# Autodesk Inventor assembly: LM2596 DC-DC Buck Converter Module
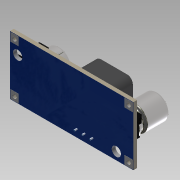
[picture p0: Inventor's stored thumbnail of the model, 180x180]
Saved by Autodesk Inventor 2019 (Build 230136000, 136)
## iProperties
Created: 2019-03-04
Part Number: LM2596 DC-DC Buck Converter Module
Document SubType Name: Assembly
Designer: ZEUSLAP
Author: ZEUSLAP
## Documents named in this file (11)
- C:\Users\Luis Pujol\Desktop\AURA MODELADO\ELECTRONICA\AURA ELECTRONICA\LM2596 DC-DC Buck Converter Module.iam
- LM2596 DC-DC Buck Converter Module.iam
- C:\Users\Luis Pujol\Dropbox\TRABAJO\DISEÑO MECANICO Y PRESUPUESTOS\CAJAS PROYECTOS\PROYECTO 1\LM2596\parts\trimpot.ipt
- C:\Users\Luis Pujol\Dropbox\TRABAJO\DISEÑO MECANICO Y PRESUPUESTOS\CAJAS PROYECTOS\PROYECTO 1\LM2596\parts\board.ipt
- C:\Users\Luis Pujol\Dropbox\TRABAJO\DISEÑO MECANICO Y PRESUPUESTOS\CAJAS PROYECTOS\PROYECTO 1\LM2596\parts\capacitor.ipt
- C:\Users\Luis Pujol\Dropbox\TRABAJO\DISEÑO MECANICO Y PRESUPUESTOS\CAJAS PROYECTOS\PROYECTO 1\LM2596\parts\CAPSMD220-35.ipt
- C:\Users\Luis Pujol\Dropbox\TRABAJO\DISEÑO MECANICO Y PRESUPUESTOS\CAJAS PROYECTOS\PROYECTO 1\LM2596\parts\Diode SMA.ipt
- C:\Users\Luis Pujol\Dropbox\TRABAJO\DISEÑO MECANICO Y PRESUPUESTOS\CAJAS PROYECTOS\PROYECTO 1\LM2596\parts\inductor.ipt
- C:\Users\Luis Pujol\Dropbox\TRABAJO\DISEÑO MECANICO Y PRESUPUESTOS\CAJAS PROYECTOS\PROYECTO 1\LM2596\parts\lm2596.ipt
- C:\Users\Luis Pujol\Dropbox\TRABAJO\DISEÑO MECANICO Y PRESUPUESTOS\CAJAS PROYECTOS\PROYECTO 1\LM2596\parts\resistor.ipt
- C:\Users\Luis Pujol\Dropbox\TRABAJO\DISEÑO MECANICO Y PRESUPUESTOS\CAJAS PROYECTOS\PROYECTO 1\LM2596\parts\solder_hole.ipt
## Components (13 placed, 9 different names)
1. board:1 — Mate:1, Mate:2, Mate:3, Mate:4, Mate:5, Mate:6, Mate:7, Mate:8, Mate:9, Mate:10, Angle:1, Mate:11, Angle:2, Mate:12, Angle:3, Mate:13, Angle:4, Angle:5, Angle:6, Mate:14, Mate:15, Mate:16, Mate:17, Mate:18, Mate:19, Mate:20, Mate:21, Mate:22, Mate:28, Mate:29
2. capacitor:1 — Mate:7, Angle:5, Mate:30, Mate:31
3. CAPSMD220-35:1 — Mate:3, Angle:3, Mate:13, Mate:28, Mate:31
4. Diode SMA:1 — Mate:5, Angle:4, Mate:22, Mate:23
5. inductor:1 — Mate:2, Mate:26, Mate:27, Mate:30
6. lm2596:1 — Mate:1, Angle:1, Mate:11, Mate:24, Mate:25, Mate:27
7. resistor:1 — Mate:8, Angle:6, Mate:29, Flush:1
8. trimpot:1 — Mate:6, Angle:2, Mate:12, Mate:25, Mate:26, Flush:1
9. CAPSMD220-35:2 — Mate:4, Mate:9, Mate:10, Mate:23, Mate:24
10. solder_hole:1 — Mate:18, Mate:19
11. solder_hole:2 — Mate:14, Mate:15
12. solder_hole:3 — Mate:16, Mate:17
13. solder_hole:4 — Mate:20, Mate:21
## Relationships (38: Mate 31, Angle 6, Flush 1)
- Mate:1: board:1 ↔ lm2596:1
- Mate:2: board:1 ↔ inductor:1
- Mate:3: board:1 ↔ CAPSMD220-35:1
- Mate:4: board:1 ↔ CAPSMD220-35:2
- Mate:5: board:1 ↔ Diode SMA:1
- Mate:6: board:1 ↔ trimpot:1
- Mate:7: board:1 ↔ capacitor:1
- Mate:8: board:1 ↔ resistor:1
- Mate:9: board:1 ↔ CAPSMD220-35:2
- Mate:10: board:1 ↔ CAPSMD220-35:2
- Angle:1 (0 deg): board:1 ↔ lm2596:1
- Mate:11: board:1 ↔ lm2596:1
- Angle:2 (-90 deg): board:1 ↔ trimpot:1
- Mate:12: board:1 ↔ trimpot:1
- Angle:3 (0 deg): board:1 ↔ CAPSMD220-35:1
- Mate:13: board:1 ↔ CAPSMD220-35:1
- Angle:4 (180 deg): board:1 ↔ Diode SMA:1
- Angle:5 (90 deg): board:1 ↔ capacitor:1
- Angle:6 (0 deg): board:1 ↔ resistor:1
- Mate:14: board:1 ↔ solder_hole:2
- Mate:15: board:1 ↔ solder_hole:2
- Mate:16: board:1 ↔ solder_hole:3
- Mate:17: board:1 ↔ solder_hole:3
- Mate:18: board:1 ↔ solder_hole:1
- Mate:19: board:1 ↔ solder_hole:1
- Mate:20: board:1 ↔ solder_hole:4
- Mate:21: board:1 ↔ solder_hole:4
- Mate:22 (3.5 mm): board:1 ↔ Diode SMA:1
- Mate:23 (2 mm): Diode SMA:1 ↔ CAPSMD220-35:2
- Mate:24 (0.5 mm): lm2596:1 ↔ CAPSMD220-35:2
- Mate:25 (0.5 mm): lm2596:1 ↔ trimpot:1
- Mate:26 (0.5 mm): inductor:1 ↔ trimpot:1
- Mate:27 (0.3 mm): inductor:1 ↔ lm2596:1
- Mate:28 (6 mm): board:1 ↔ CAPSMD220-35:1
- Mate:29 (1.5 mm): board:1 ↔ resistor:1
- Flush:1 (-2 mm): resistor:1 ↔ trimpot:1
- Mate:30 (2 mm): capacitor:1 ↔ inductor:1
- Mate:31 (1 mm): capacitor:1 ↔ CAPSMD220-35:1
